# Autodesk Inventor assembly: 393 Motor
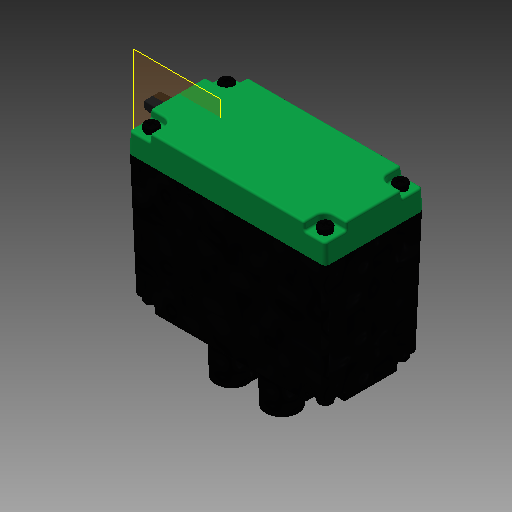
[picture p0: Inventor's stored thumbnail of the model, 512x512]
Saved by Autodesk Inventor 2019 (Build 230136000, 136)
## iProperties
Created: 2012-04-13
Part Number: 393 Motor
Document SubType Name: Assembly
Designer: Phillip
Author: Phillip
## Documents named in this file (8)
- C:\Users\Taran Mayer\Desktop\VEX Parts Library 2016\Imperial\Motion\393 Motor.iam
- C:\Users\Taran Mayer\Desktop\VEX Parts Library 2016\Imperial\Motion\Components\SPPM206-0150BO.ipt
- C:\Users\Taran Mayer\Desktop\VEX Parts Library 2016\Imperial\Motion\Components\276-2177-002 Rev1.ipt
- C:\Users\Taran Mayer\Desktop\VEX Parts Library 2016\Imperial\Motion\Components\276-2177-003 Rev1.ipt
- C:\Users\Taran Mayer\Desktop\VEX Parts Library 2016\Imperial\Motion\Components\276-2177-018 Rev1.ipt
- C:\Users\Taran Mayer\Desktop\VEX Parts Library 2016\Imperial\Motion\Components\276-2177-019 Rev1.ipt
- C:\Users\Taran Mayer\Desktop\VEX Parts Library 2016\Imperial\Motion\Components\276-2177-008 Rev1.ipt
- C:\Users\Taran Mayer\Desktop\VEX Parts Library 2016\Imperial\Motion\Components\276-2177-001 Rev1.ipt
## Components (15 placed, 7 different names)
1. 276-2177-002 Rev1:1 — Mate:3, Flush:4, Mate:4, Mate:6, Mate:7, Mate:8
2. SPPM206-0150BO:1 — Insert:3
3. 276-2177-003 Rev1:1 — Insert:1, Insert:2, Insert:3, Insert:4, Flush:3, Mate:3, Flush:4, Mate:4, Mate:5, Mate:9, Mate:10, Flush:5, Flush:11
4. SPPM206-0150BO:2 — Insert:6, Mate:7
5. SPPM206-0150BO:3 — Insert:5
6. 276-2177-018 Rev1:1
7. SPPM206-0150BO:4 — Insert:2
8. 276-2177-019 Rev1:1 — Mate:10, Flush:11
9. 276-2177-019 Rev1:2 — Mate:9, Flush:5
10. SPPM206-0150BO:5 — Insert:4
11. SPPM206-0150BO:6 — Insert:8
12. SPPM206-0150BO:7 — Insert:1
13. 276-2177-008 Rev1:1 — Flush:3, Mate:5
14. 276-2177-001 Rev1:1 — Insert:5, Insert:6, Insert:7, Insert:8, Mate:6, Mate:8
15. SPPM206-0150BO:8 — Insert:7
## Relationships (20: Insert 8, Mate 8, Flush 4)
- Insert:1: 276-2177-003 Rev1:1 ↔ SPPM206-0150BO:7
- Insert:2: 276-2177-003 Rev1:1 ↔ SPPM206-0150BO:4
- Insert:3: SPPM206-0150BO:1 ↔ 276-2177-003 Rev1:1
- Insert:4: 276-2177-003 Rev1:1 ↔ SPPM206-0150BO:5
- Insert:5: SPPM206-0150BO:3 ↔ 276-2177-001 Rev1:1
- Insert:6: SPPM206-0150BO:2 ↔ 276-2177-001 Rev1:1
- Insert:7: 276-2177-001 Rev1:1 ↔ SPPM206-0150BO:8
- Insert:8: SPPM206-0150BO:6 ↔ 276-2177-001 Rev1:1
- Flush:3 (-0.0508 mm): 276-2177-003 Rev1:1 ↔ 276-2177-008 Rev1:1
- Mate:3: 276-2177-002 Rev1:1 ↔ 276-2177-003 Rev1:1
- Flush:4: 276-2177-002 Rev1:1 ↔ 276-2177-003 Rev1:1
- Mate:4: 276-2177-002 Rev1:1 ↔ 276-2177-003 Rev1:1
- Mate:5: 276-2177-003 Rev1:1 ↔ 276-2177-008 Rev1:1
- Mate:6: 276-2177-002 Rev1:1 ↔ 276-2177-001 Rev1:1
- Mate:7: 276-2177-002 Rev1:1 ↔ SPPM206-0150BO:2
- Mate:8: 276-2177-002 Rev1:1 ↔ 276-2177-001 Rev1:1
- Mate:9: 276-2177-003 Rev1:1 ↔ 276-2177-019 Rev1:2
- Mate:10: 276-2177-003 Rev1:1 ↔ 276-2177-019 Rev1:1
- Flush:5 (0.7366 mm): 276-2177-003 Rev1:1 ↔ 276-2177-019 Rev1:2
- Flush:11 (0.7366 mm): 276-2177-003 Rev1:1 ↔ 276-2177-019 Rev1:1
